# Autodesk Inventor assembly: ass-b
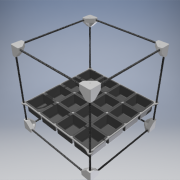
[picture p0: Inventor's stored thumbnail of the model, 180x180]
Saved by Autodesk Inventor 2017 (Build 210142000, 142)
## iProperties
Created: 2019-02-09
Part Number: ass-b
Document SubType Name: Assembly
Designer: felix
Author: felix
## Documents named in this file (7)
- C:\Users\felix\OneDrive\Documentos\Git\Garatéa E-3\probe-b.iam
- C:\Users\felix\OneDrive\Documentos\Git\Garatéa E-3\probe-b\b-base.ipt
- C:\Users\felix\OneDrive\Documentos\Git\Garatéa E-3\sats\big_sat.ipt
- C:\Users\felix\OneDrive\Documentos\Git\Garatéa E-3\probe-b\b-carbon_pipe.ipt
- C:\Users\felix\OneDrive\Documentos\Git\Garatéa E-3\probe-b\b-connector.ipt
- C:\Users\felix\OneDrive\Documentos\Git\Garatéa E-3\probe-b\b-connector_MIR.ipt
- C:\Users\felix\OneDrive\Documentos\Git\Garatéa E-3\probe-b\b-carbon_pipe_MIR.ipt
## Components (37 placed, 6 different names)
1. b-base:1 — Mate:1, Mate:2, Mate:3, Mate:10
2. big_sat:1 — Mate:1, Mate:2, Mate:3
3. big_sat:2
4. big_sat:3
5. big_sat:4
6. big_sat:5
7. big_sat:6
8. big_sat:7
9. big_sat:8
10. big_sat:9
11. big_sat:10
12. big_sat:11
13. big_sat:12
14. big_sat:13
15. big_sat:14
16. big_sat:15
17. big_sat:16
18. b-carbon_pipe_MIR:1 — Mate:8, Mate:9
19. b-connector_MIR:1 — Mate:8, Mate:9, Mate:11, Mate:12
20. b-carbon_pipe:1 — Mate:4, Mate:5, Mate:10, Mate:11, Mate:12
21. b-connector:1 — Mate:4, Mate:5, Mate:6, Mate:7
22. b-carbon_pipe:2 — Mate:6, Mate:7
23. b-carbon_pipe_MIR:2
24. b-connector_MIR:2
25. b-carbon_pipe:3
26. b-connector:2
27. b-carbon_pipe:4
28. b-carbon_pipe_MIR:3
29. b-connector_MIR:3
30. b-carbon_pipe:5
31. b-connector:3
32. b-carbon_pipe:6
33. b-carbon_pipe_MIR:4
34. b-connector_MIR:4
35. b-carbon_pipe:7
36. b-connector:4
37. b-carbon_pipe:8
## Component patterns: (16 elements, first: big_sat:1), (4 elements, first: b-carbon_pipe_MIR:1 + b-connector_MIR:1 + b-carbon_pipe:1 + b-connector:1 + b-carbon_pipe:2)
## Relationships (12: Mate 12)
- Mate:1: b-base:1 ↔ big_sat:1
- Mate:2: b-base:1 ↔ big_sat:1
- Mate:3: b-base:1 ↔ big_sat:1
- Mate:4: b-carbon_pipe:1 ↔ b-connector:1
- Mate:5: b-carbon_pipe:1 ↔ b-connector:1
- Mate:6: b-connector:1 ↔ b-carbon_pipe:2
- Mate:7: b-connector:1 ↔ b-carbon_pipe:2
- Mate:8: b-carbon_pipe_MIR:1 ↔ b-connector_MIR:1
- Mate:9: b-carbon_pipe_MIR:1 ↔ b-connector_MIR:1
- Mate:10: b-base:1 ↔ b-carbon_pipe:1
- Mate:11: b-connector_MIR:1 ↔ b-carbon_pipe:1
- Mate:12: b-connector_MIR:1 ↔ b-carbon_pipe:1
